# Autodesk Inventor assembly: fischer price 20-1 reduction
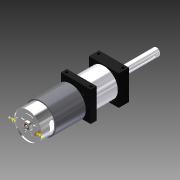
[picture p0: Inventor's stored thumbnail of the model, 180x180]
Saved by Autodesk Inventor 2011 (Build 150239000, 239)
## iProperties
Created: 2010-02-09
Part Number: fischer price 20-1 reduction
Document SubType Name: Assembly
Designer: a
Author: a
## Documents named in this file (3)
- R:\2012\Inventor\vkop\All_Motors\fischer price 20-1 reduction.iam
- R:\2012\Inventor\vkop\All_Motors\banebot 20-1 fischer price.ipt
- R:\2012\Inventor\vkop\All_Motors\Motors_BaneBots_RS-550.ipt
## Components (2 placed, 2 different names)
1. banebot 20-1 fischer price:1 — Mate:1, Mate:2
2. Motors_BaneBots_RS-550:1 — Mate:1, Mate:2
## Relationships (2: Mate 2)
- Mate:1: banebot 20-1 fischer price:1 ↔ Motors_BaneBots_RS-550:1
- Mate:2: banebot 20-1 fischer price:1 ↔ Motors_BaneBots_RS-550:1
